# Autodesk Inventor assembly: b1
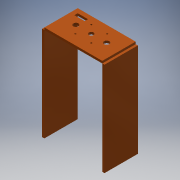
[picture p0: Inventor's stored thumbnail of the model, 180x180]
Saved by Autodesk Inventor 2017 (Build 210142000, 142)
## iProperties
Created: 2015-10-11
Part Number: b1
Document SubType Name: Assembly
Designer: daniel
Author: daniel
## Documents named in this file (3)
- C:\Users\daniel\Documents\GitHub\cardboard-stage-metric\stage\b1.iam
- C:\Users\daniel\Documents\GitHub\cardboard-stage-metric\stage\b1b.ipt
- C:\Users\daniel\Documents\GitHub\cardboard-stage-metric\stage\b1a.ipt
## Components (3 placed, 2 different names)
1. b1a:1 — Flush:3, Mate:3, Flush:5, Mate:4, Mate:5, Mate:6
2. b1b:1 — Flush:3, Mate:3, Flush:4, Flush:6, Mate:6
3. b1b:2 — Flush:4, Flush:5, Flush:6, Mate:4, Mate:5
## Relationships (8: Flush 4, Mate 4)
- Flush:3: b1a:1 ↔ b1b:1
- Mate:3: b1a:1 ↔ b1b:1
- Flush:4: b1b:1 ↔ b1b:2
- Flush:5: b1a:1 ↔ b1b:2
- Flush:6: b1b:1 ↔ b1b:2
- Mate:4: b1a:1 ↔ b1b:2
- Mate:5: b1a:1 ↔ b1b:2
- Mate:6: b1a:1 ↔ b1b:1
